# Autodesk Inventor assembly: MIR_HbIndexFinger01ForChild
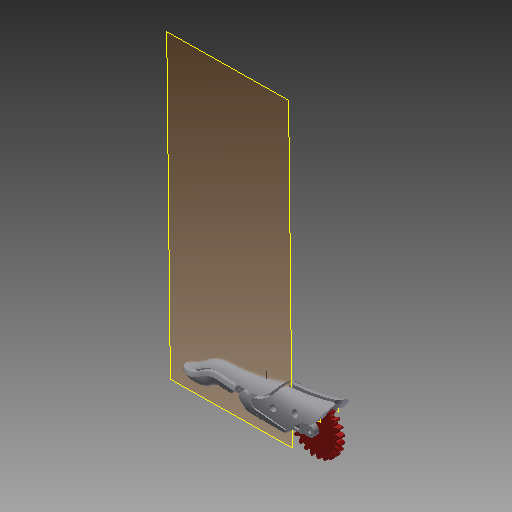
[picture p0: Inventor's stored thumbnail of the model, 512x512]
Saved by Autodesk Inventor 2018.1 (Build 221171000, 171)
## iProperties
Part Number: MIR_HbIndexFinger01ForChild
Material: 一般
Document SubType Name: Assembly
Designer: sktom
Author: sktom
## Documents named in this file (11)
- D:\CloudStrage\OneDrive\CAD\MAJ\hackberry\HACKberry-hardware\3D_69%inlength\Inventor\HbHandForChild\HbIndexFinger01ForChild\MIR_HbIndexFinger01ForChild.iam
- D:\CloudStrage\OneDrive\CAD\MAJ\hackberry\HACKberry-hardware\3D_69%inlength\Inventor\HbHandForChild\HbIndexFinger01ForChild\MIR_HbIndexMiddle-DistalPhalanx02ForChild.ipt
- D:\CloudStrage\OneDrive\CAD\MAJ\hackberry\HACKberry-hardware\3D_69%inlength\Inventor\HbHandForChild\HbIndexFinger01ForChild\MIR_HbIndexCouplerLink02ForChild.ipt
- D:\CloudStrage\OneDrive\CAD\MAJ\hackberry\HACKberry-hardware\3D_69%inlength\Inventor\HbHandForChild\HbIndexFinger01ForChild\MIR_HbIndexCouplerLinkCover02ForChild.ipt
- D:\CloudStrage\OneDrive\CAD\MAJ\hackberry\HACKberry-hardware\3D_69%inlength\Inventor\HbHandForChild\HbIndexFinger01ForChild\MIR_HbIndexProximalPhalanx03ForChild.ipt
- D:\CloudStrage\OneDrive\CAD\MAJ\hackberry\HACKberry-hardware\3D_69%inlength\Inventor\HbHandForChild\HbIndexFinger01ForChild\MIR_HbIndexProximalPhalanxCover02ForChild.ipt
- D:\CloudStrage\OneDrive\CAD\MAJ\hackberry\HACKberry-hardware\3D_69%inlength\Inventor\HbHandForChild\HbIndexFinger01ForChild\MIR_HbIndexReleaseLever02ForChild.ipt
- D:\CloudStrage\OneDrive\CAD\MAJ\hackberry\HACKberry-hardware\3D_69%inlength\Inventor\HbHandForChild\HbIndexFinger01ForChild\MIR_Spur Gear (24 teeth).ipt
- D:\CloudStrage\OneDrive\CAD\MAJ\hackberry\HACKberry-hardware\3D_69%inlength\Inventor\HbHandForChild\HbIndexFinger01ForChild\MIR_shaft_phi1.5_l6.ipt
- D:\CloudStrage\OneDrive\CAD\MAJ\hackberry\HACKberry-hardware\3D_69%inlength\Inventor\HbHandForChild\MIR_TOS 0.3-3-270ﾟ-3.ipt
- D:\CloudStrage\OneDrive\CAD\MAJ\hackberry\HACKberry-hardware\3D_69%inlength\Inventor\HbHandForChild\HbIndexFinger01ForChild\MIR_bolt_M1.4L6.ipt
## Components (16 placed, 10 different names)
1. MIR_HbIndexMiddle-DistalPhalanx02ForChild:1 — 挿入:20, 挿入:18, 挿入:17, 円柱状:3, 円柱状:4
2. MIR_HbIndexCouplerLink02ForChild:1 — 挿入:3, 挿入:2, 挿入:14
3. MIR_HbIndexCouplerLinkCover02ForChild:1 — 挿入:20, 挿入:3, 挿入:2, 挿入:21, 挿入:22
4. MIR_HbIndexProximalPhalanx03ForChild:1 — 挿入:16, 挿入:15, 挿入:23, 挿入:24
5. MIR_HbIndexProximalPhalanxCover02ForChild:1 — 挿入:18, 挿入:16, 挿入:15, 挿入:19, メイト:1, 円柱状:3, 円柱状:5
6. MIR_HbIndexReleaseLever02ForChild:1 — 挿入:19, 回転:1
7. MIR_Spur Gear (24 teeth):1 — メイト:1, 円柱状:5, 円柱状:6
8. MIR_shaft_phi1.5_l6:1 — 挿入:17, フラッシュ:1
9. MIR_shaft_phi1.5_l6:2 — フラッシュ:1, 円柱状:4
10. MIR_shaft_phi1.5_l6:3 — 回転:1
11. MIR_shaft_phi1.5_l6:4 — 挿入:14, 円柱状:6
12. MIR_TOS 0.3-3-270ﾟ-3:1
13. MIR_bolt_M1.4L6:1 — 挿入:21
14. MIR_bolt_M1.4L6:2 — 挿入:22
15. MIR_bolt_M1.4L6:3 — 挿入:23
16. MIR_bolt_M1.4L6:4 — 挿入:24
## Relationships (20: Insert 13, CylindricalJoint 4, Mate 1, Flush 1, RevoluteJoint 1)
- 挿入:20 [Insert] (0.1 mm): MIR_HbIndexMiddle-DistalPhalanx02ForChild:1 ↔ MIR_HbIndexCouplerLinkCover02ForChild:1
- 挿入:3 [Insert]: MIR_HbIndexCouplerLink02ForChild:1 ↔ MIR_HbIndexCouplerLinkCover02ForChild:1
- 挿入:2 [Insert]: MIR_HbIndexCouplerLink02ForChild:1 ↔ MIR_HbIndexCouplerLinkCover02ForChild:1
- 挿入:18 [Insert] (0.025 mm): MIR_HbIndexMiddle-DistalPhalanx02ForChild:1 ↔ MIR_HbIndexProximalPhalanxCover02ForChild:1
- 挿入:16 [Insert]: MIR_HbIndexProximalPhalanx03ForChild:1 ↔ MIR_HbIndexProximalPhalanxCover02ForChild:1
- 挿入:15 [Insert]: MIR_HbIndexProximalPhalanx03ForChild:1 ↔ MIR_HbIndexProximalPhalanxCover02ForChild:1
- 挿入:19 [Insert] (0.4 mm): MIR_HbIndexProximalPhalanxCover02ForChild:1 ↔ MIR_HbIndexReleaseLever02ForChild:1
- メイト:1 [Mate] (0.1 mm): MIR_HbIndexProximalPhalanxCover02ForChild:1 ↔ MIR_Spur Gear (24 teeth):1
- 挿入:17 [Insert] (-0.8 mm): MIR_HbIndexMiddle-DistalPhalanx02ForChild:1 ↔ MIR_shaft_phi1.5_l6:1
- フラッシュ:1 [Flush]: MIR_shaft_phi1.5_l6:1 ↔ MIR_shaft_phi1.5_l6:2
- 挿入:14 [Insert] (-2 mm): MIR_HbIndexCouplerLink02ForChild:1 ↔ MIR_shaft_phi1.5_l6:4
- 挿入:21 [Insert]: MIR_HbIndexCouplerLinkCover02ForChild:1 ↔ MIR_bolt_M1.4L6:1
- 挿入:22 [Insert]: MIR_HbIndexCouplerLinkCover02ForChild:1 ↔ MIR_bolt_M1.4L6:2
- 挿入:23 [Insert]: MIR_HbIndexProximalPhalanx03ForChild:1 ↔ MIR_bolt_M1.4L6:3
- 挿入:24 [Insert]: MIR_HbIndexProximalPhalanx03ForChild:1 ↔ MIR_bolt_M1.4L6:4
- 円柱状:3 [CylindricalJoint]: MIR_HbIndexMiddle-DistalPhalanx02ForChild:1 ↔ MIR_HbIndexProximalPhalanxCover02ForChild:1
- 円柱状:5 [CylindricalJoint]: MIR_HbIndexProximalPhalanxCover02ForChild:1 ↔ MIR_Spur Gear (24 teeth):1
- 円柱状:4 [CylindricalJoint]: MIR_HbIndexMiddle-DistalPhalanx02ForChild:1 ↔ MIR_shaft_phi1.5_l6:2
- 回転:1 [RevoluteJoint]: MIR_HbIndexReleaseLever02ForChild:1 ↔ MIR_shaft_phi1.5_l6:3
- 円柱状:6 [CylindricalJoint]: MIR_Spur Gear (24 teeth):1 ↔ MIR_shaft_phi1.5_l6:4
